# Autodesk Inventor assembly: finalass
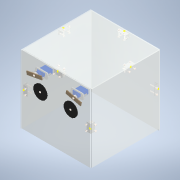
[picture p0: Inventor's stored thumbnail of the model, 180x180]
Saved by Autodesk Inventor 2021 (Build 250183000, 183)
## iProperties
Created: 2023-06-07
Part Number: finalass
Document SubType Name: Assembly
Designer: shrus
Author: shrus
## Documents named in this file (13)
- C:\Users\shrus\Desktop\finalass.iam
- C:\Users\shrus\Documents\facef.ipt
- C:\Users\shrus\Documents\Assembly servo2.iam
- C:\Users\shrus\Documents\Ass eyebrow.iam
- C:\Users\shrus\Documents\assembly servo1.iam
- C:\Users\shrus\Documents\m3-25mm.ipt
- C:\Users\shrus\Documents\M3 Nut.ipt
- C:\Users\shrus\Documents\eye ass.iam
- C:\Users\shrus\Documents\Hinge angle.ipt
- C:\Users\shrus\Documents\Hing ass.iam
- C:\Users\shrus\Documents\m3-6mm.ipt
- C:\Users\shrus\Documents\leftright.ipt
- C:\Users\shrus\Documents\m3-16mm.ipt
## Components (44 placed, 12 different names)
1. facef:1 — Mate:1, Mate:2, Mate:3, Mate:4, Mate:5, Mate:6, Mate:11, Mate:12, Mate:13, Mate:14, Mate:15, Mate:16, Mate:17, Mate:18, Mate:36, Mate:37, Mate:40, Mate:41
2. Assembly servo2:1 [sub-assembly] — Mate:1, Mate:7, Mate:8
3. Ass eyebrow:1 [sub-assembly] — Mate:12
4. Ass eyebrow:2 [sub-assembly] — Mate:11
5. assembly servo1:1 [sub-assembly] — Mate:2, Mate:9, Mate:10
6. m3-25mm:2 — Mate:6
7. m3-25mm:3 — Mate:3
8. m3-25mm:4 — Mate:4
9. m3-25mm:5 — Mate:5
10. M3 Nut:1 — Mate:7
11. M3 Nut:2 — Mate:8
12. M3 Nut:3 — Mate:10
13. M3 Nut:4 — Mate:9
14. eye ass:1 [sub-assembly] — Mate:14
15. eye ass:2 [sub-assembly] — Mate:13
16. M3 Nut:5 — Mate:15
17. M3 Nut:6 — Mate:16
18. Hing ass:1 [sub-assembly] — Mate:19, Mate:22, Mate:23, Mate:29, Mate:30, Mate:31, Mate:34, Mate:35
19. M3 Nut:7 — Mate:21
20. M3 Nut:8 — Mate:20
21. m3-6mm:1 — Mate:17, Mate:19, Mate:21
22. m3-6mm:2 — Mate:18, Mate:20
23. leftright:1 — Mate:22, Mate:23, Mate:24, Mate:25, Mate:38, Mate:39
24. leftright:2 — Mate:26, Mate:27
25. m3-16mm:1 — Mate:24
26. m3-16mm:2 — Mate:25
27. m3-16mm:3 — Mate:26, Mate:28
28. m3-16mm:4 — Mate:27
29. M3 Nut:9 — Mate:29
30. M3 Nut:10 — Mate:28
31. m3-16mm:5 — Mate:31
32. m3-16mm:6 — Mate:30
33. Hing ass:3 [sub-assembly] — Mate:32, Mate:33
34. m3-16mm:8 — Mate:32
35. m3-16mm:9 — Mate:33
36. m3-16mm:10 — Mate:34
37. m3-16mm:11 — Mate:35
38. Hinge angle:7
39. m3-16mm:12 — Mate:37
40. m3-16mm:13 — Mate:36
41. m3-16mm:14 — Mate:39
42. m3-16mm:15 — Mate:38
43. m3-16mm:16 — Mate:40
44. m3-16mm:17 — Mate:41
## Relationships (41: Mate 41)
- Mate:1: facef:1 ↔ Assembly servo2:1
- Mate:2: facef:1 ↔ assembly servo1:1
- Mate:3: facef:1 ↔ m3-25mm:3
- Mate:4: facef:1 ↔ m3-25mm:4
- Mate:5: facef:1 ↔ m3-25mm:5
- Mate:6: facef:1 ↔ m3-25mm:2
- Mate:7: Assembly servo2:1 ↔ M3 Nut:1
- Mate:8: Assembly servo2:1 ↔ M3 Nut:2
- Mate:9: assembly servo1:1 ↔ M3 Nut:4
- Mate:10: assembly servo1:1 ↔ M3 Nut:3
- Mate:11: facef:1 ↔ Ass eyebrow:2
- Mate:12: facef:1 ↔ Ass eyebrow:1
- Mate:13: facef:1 ↔ eye ass:2
- Mate:14: facef:1 ↔ eye ass:1
- Mate:15: facef:1 ↔ M3 Nut:5
- Mate:16: facef:1 ↔ M3 Nut:6
- Mate:17: facef:1 ↔ m3-6mm:1
- Mate:18: facef:1 ↔ m3-6mm:2
- Mate:19: Hing ass:1 ↔ m3-6mm:1
- Mate:20: M3 Nut:8 ↔ m3-6mm:2
- Mate:21: M3 Nut:7 ↔ m3-6mm:1
- Mate:22: Hing ass:1 ↔ leftright:1
- Mate:23: Hing ass:1 ↔ leftright:1
- Mate:24: leftright:1 ↔ m3-16mm:1
- Mate:25: leftright:1 ↔ m3-16mm:2
- Mate:26: leftright:2 ↔ m3-16mm:3
- Mate:27: leftright:2 ↔ m3-16mm:4
- Mate:28: m3-16mm:3 ↔ M3 Nut:10
- Mate:29: Hing ass:1 ↔ M3 Nut:9
- Mate:30: Hing ass:1 ↔ m3-16mm:6
- Mate:31: Hing ass:1 ↔ m3-16mm:5
- Mate:32: Hing ass:3 ↔ m3-16mm:8
- Mate:33: Hing ass:3 ↔ m3-16mm:9
- Mate:34: Hing ass:1 ↔ m3-16mm:10
- Mate:35: Hing ass:1 ↔ m3-16mm:11
- Mate:36: facef:1 ↔ m3-16mm:13
- Mate:37: facef:1 ↔ m3-16mm:12
- Mate:38: leftright:1 ↔ m3-16mm:15
- Mate:39: leftright:1 ↔ m3-16mm:14
- Mate:40: facef:1 ↔ m3-16mm:16
- Mate:41: facef:1 ↔ m3-16mm:17
